# Autodesk Inventor assembly: robotArmWithWormGearBox
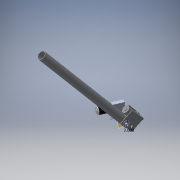
[picture p0: Inventor's stored thumbnail of the model, 180x180]
Saved by Autodesk Inventor 2018.2 (Build 222227000, 227)
## iProperties
Created: 2017-04-29
Part Number: robotArmWithWormGearBox
Document SubType Name: Assembly
Designer: steele
Author: steele
## Documents named in this file (11)
- D:\snobotics\CAD-Development\robSteele\2018-FRC\GripperArm\robotArmWithWormGearBox.iam
- D:\snobotics\CAD-Development\robSteele\SnoBotics2017\Arm\am-0077a-500 Key Hub r2.ipt
- D:\snobotics\CAD-Development\robSteele\SnoBotics2017\Arm\am-0917+WormBox.iam
- D:\snobotics\CAD-Development\robSteele\SnoBotics2017\Arm\am-2099+Collar+Clamp,+0.5''+Bore,+Aluminum.iam
- D:\snobotics\CAD-Development\robSteele\SnoBotics2017\Arm\robotArmWithWormGearBox\Design Accelerator\Bolted Connection1.iam
- D:\snobotics\CAD-Development\robSteele\SnoBotics2017\Arm\robotArmWithWormGearBox\Design Accelerator\Bolted Connection2.iam
- D:\snobotics\CAD-MfgResources\Andy-Mark\Linear Actuators\DART 12 in Actuator AM-3072a\am-3072aDART12.iam
- D:\snobotics\CAD-Development\robSteele\2018-FRC\GripperArm\supportPlateForLinearActuator.ipt
- D:\snobotics\CAD-Development\robSteele\SnoBotics2017\Arm\am-0077a-500 Key Hub r2_MIR.ipt
- D:\snobotics\CAD-Development\robSteele\2018-FRC\GripperArm\supportPlateForLinearActuator_MIR.ipt
- D:\snobotics\CAD-Development\robSteele\2018-FRC\PVC Pipe\2_5-inch schedule 40 forArm.ipt
## Components (10 placed, 9 different names)
1. am-0917+WormBox:1 [sub-assembly] — Insert:6, Mate:4, Mate:5
2. am-0077a-500 Key Hub r2:1 — Insert:6, Insert:7, Insert:8, Insert:9, Flush:3
3. am-2099+Collar+Clamp,+0.5''+Bore,+Aluminum:1 [sub-assembly] — Insert:7
4. Bolted Connection:1 [sub-assembly]
5. Bolted Connection:2 [sub-assembly] — Mate:4, Mate:5
6. am-3072aDART12:1 [sub-assembly] — Mate:6, Flush:1, Flush:2, Insert:12
7. supportPlateForLinearActuator:1 — Insert:8, Insert:9, Mate:6, Flush:1, Flush:2
8. am-0077a-500 Key Hub r2_MIR:1 — Insert:10, Insert:11, Mate:7
9. supportPlateForLinearActuator_MIR:1 — Insert:10, Insert:11
10. 2_5-inch schedule 40 forArm:1 — Insert:12
## Relationships (14: Insert 7, Mate 4, Flush 3)
- Insert:6: am-0917+WormBox:1 ↔ am-0077a-500 Key Hub r2:1
- Insert:7: am-0077a-500 Key Hub r2:1 ↔ am-2099+Collar+Clamp,+0.5''+Bore,+Aluminum:1
- Mate:4: am-0917+WormBox:1 ↔ Bolted Connection:2
- Mate:5: am-0917+WormBox:1 ↔ Bolted Connection:2
- Insert:8: am-0077a-500 Key Hub r2:1 ↔ supportPlateForLinearActuator:1
- Insert:9: am-0077a-500 Key Hub r2:1 ↔ supportPlateForLinearActuator:1
- Mate:6: am-3072aDART12:1 ↔ supportPlateForLinearActuator:1
- Flush:1: am-3072aDART12:1 ↔ supportPlateForLinearActuator:1
- Flush:2: am-3072aDART12:1 ↔ supportPlateForLinearActuator:1
- Flush:3 (47.625 mm): am-0077a-500 Key Hub r2:1
- Insert:10: am-0077a-500 Key Hub r2_MIR:1 ↔ supportPlateForLinearActuator_MIR:1
- Insert:11: am-0077a-500 Key Hub r2_MIR:1 ↔ supportPlateForLinearActuator_MIR:1
- Mate:7 (34.925 mm): am-0077a-500 Key Hub r2_MIR:1
- Insert:12 (-381 mm): am-3072aDART12:1 ↔ 2_5-inch schedule 40 forArm:1
